# Autodesk Inventor assembly: battery_protection_battery-protection
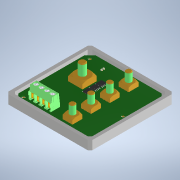
[picture p0: Inventor's stored thumbnail of the model, 180x180]
Saved by Autodesk Inventor 2020.3 (Build 243373000, 373)
## iProperties
Company: A Company
Created: 2020-07-08
Part Number: battery_protection_battery-protection
Description: KiCad electronic assembly
Document SubType Name: Assembly
Designer: OskarJohansson
Authority: Unknown
Sending System: KiCad to STEP converter
Preprocessor: Open CASCADE STEP processor 6.9
Title: battery-protection.step
Author: An Author
## Documents named in this file (11)
- C:\Users\OskarJohansson\Dropbox\Dokument\Projekt\Elita\Electrical system\Highside-Powerdistribution\hardware\cad\battery-protection\battery_protection_battery-protection.iam
- C:\Users\OskarJohansson\Dropbox\Dokument\Projekt\Elita\Electrical system\Highside-Powerdistribution\hardware\cad\battery-protection\battery_protection_Phoenix_pxc_1935187_04_PT-1-5-4-5-0-H_3D.iam
- C:\Users\OskarJohansson\Dropbox\Dokument\Projekt\Elita\Electrical system\Highside-Powerdistribution\hardware\cad\battery-protection\battery_protection_PowerPAK_SO-8L_SINGLE.iam
- C:\Users\OskarJohansson\Dropbox\Dokument\Projekt\Elita\Electrical system\Highside-Powerdistribution\hardware\cad\battery-protection\battery_protection_R_0603_1608Metric.iam
- C:\Users\OskarJohansson\Dropbox\Dokument\Projekt\Elita\Electrical system\Highside-Powerdistribution\hardware\cad\battery-protection\battery_protection_M6_7461098_rev1.iam
- C:\Users\OskarJohansson\Dropbox\Dokument\Projekt\Elita\Electrical system\Highside-Powerdistribution\hardware\cad\battery-protection\battery_protection_M5_7461383_rev1.iam
- C:\Users\OskarJohansson\Dropbox\Dokument\Projekt\Elita\Electrical system\Highside-Powerdistribution\hardware\cad\battery-protection\battery_protection_SOT-23-8.iam
- C:\Users\OskarJohansson\Dropbox\Dokument\Projekt\Elita\Electrical system\Highside-Powerdistribution\hardware\cad\battery-protection\battery_protection_LED_0603_1608Metric.iam
- C:\Users\OskarJohansson\Dropbox\Dokument\Projekt\Elita\Electrical system\Highside-Powerdistribution\hardware\cad\battery-protection\battery_protection_SOT-23.iam
- C:\Users\OskarJohansson\Dropbox\Dokument\Projekt\Elita\Electrical system\Highside-Powerdistribution\hardware\cad\battery-protection\battery_protection_COMPOUND_2.ipt
- C:\Users\OskarJohansson\Documents\GitHub\outdoor-sense\hardware\cad\enclosure\aluminium_block.ipt
## Components (25 placed, 25 different names)
1. 2 [sub-assembly]
2. 4 [sub-assembly]
3. 5 [sub-assembly]
4. 6 [sub-assembly]
5. 7 [sub-assembly]
6. 8 [sub-assembly]
7. 9 [sub-assembly]
8. 11 [sub-assembly]
9. 12 [sub-assembly]
10. 14 [sub-assembly]
11. 16 [sub-assembly]
12. 17 [sub-assembly]
13. 18 [sub-assembly]
14. 20 [sub-assembly]
15. 22 [sub-assembly]
16. 23 [sub-assembly]
17. 24 [sub-assembly]
18. 25 [sub-assembly]
19. 27 [sub-assembly]
20. 28 [sub-assembly]
21. 29 [sub-assembly]
22. 30 [sub-assembly]
23. 31 [sub-assembly]
24. 32 — Flush:1
25. aluminium_block:1 — Flush:1
## Relationships (1: Flush 1)
- Flush:1: 32 ↔ aluminium_block:1
